# Autodesk Inventor assembly: Assembly E
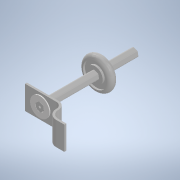
[picture p0: Inventor's stored thumbnail of the model, 180x180]
Saved by Autodesk Inventor 2021 (Build 250183000, 183)
## iProperties
Created: 2020-12-11
Part Number: Assembly E
Document SubType Name: Assembly
Designer: aidan
Author: aidan
## Documents named in this file (5)
- C:\Users\aidan\Desktop\T3 Robotics\CAD\Assembly E.iam
- C:\Users\aidan\Desktop\T3 Robotics\CAD\Wheel v3 EDD.ipt
- C:\Users\aidan\Desktop\T3 Robotics\CAD\Bearing for THUNDER.ipt
- C:\Users\aidan\Desktop\T3 Robotics\CAD\Shaped Metal Thing v1 EDD.ipt
- C:\Users\aidan\Desktop\T3 Robotics\CAD\Thundershaft v1 EDD.ipt
## Components (4 placed, 4 different names)
1. Wheel v3 EDD:1 — Mate:2, Mate:3, Flush:2
2. Bearing for THUNDER:1 — Mate:1, Flush:1, Mate:4, Mate:5
3. Shaped Metal Thing v1 EDD:1 — Mate:4, Mate:5
4. Thundershaft v1 EDD:1 — Mate:1, Flush:1, Mate:2, Mate:3, Flush:2
## Relationships (7: Mate 5, Flush 2)
- Mate:1: Bearing for THUNDER:1 ↔ Thundershaft v1 EDD:1
- Flush:1: Bearing for THUNDER:1 ↔ Thundershaft v1 EDD:1
- Mate:2: Wheel v3 EDD:1 ↔ Thundershaft v1 EDD:1
- Mate:3: Wheel v3 EDD:1 ↔ Thundershaft v1 EDD:1
- Mate:4: Bearing for THUNDER:1 ↔ Shaped Metal Thing v1 EDD:1
- Mate:5: Bearing for THUNDER:1 ↔ Shaped Metal Thing v1 EDD:1
- Flush:2 (50.8 mm): Wheel v3 EDD:1 ↔ Thundershaft v1 EDD:1
